# Autodesk Inventor assembly: XY Joint Left (Tulip)
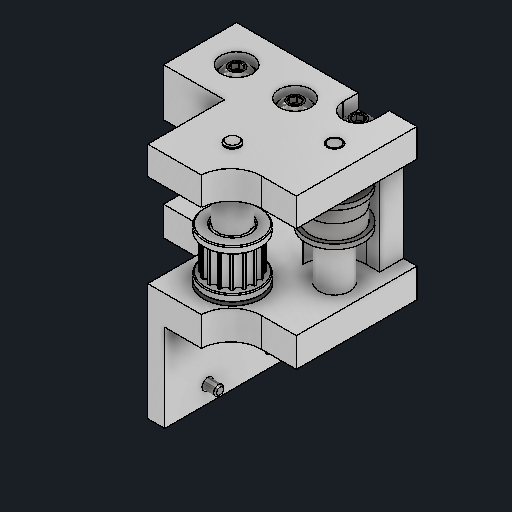
[picture p0: Inventor's stored thumbnail of the model, 512x512]
Saved by Autodesk Inventor 2026.1 (Build 301233020, 233B)
## iProperties
Created: 2025-05-24
Part Number: XY Joint Left (Tulip)
Document SubType Name: Assembly
Designer: Joshua Eah
Author: Joshua Eah
## Documents named in this file (10)
- C:\Users\JoshuaEah\Documents\GitHub\Voron-0\CAD\Tulip - Machined Parts\XY Joints\XY Joint Right\XY Joint Right (Tulip).iam
- C:\Users\JoshuaEah\Documents\GitHub\Voron-0\CAD\Tulip - Machined Parts\XY Joints\XY Joint Right\XY Joint Right Upper (Tulip).ipt
- C:\Users\JoshuaEah\Documents\GitHub\Voron-0\CAD\Tulip - Machined Parts\XY Joints\XY Joint Right\XY Joint Right Lower (Tulip).ipt
- C:\Users\JoshuaEah\Documents\GitHub\Voron-0\CAD\Master Assembly\Hardware\M3x6 BHCS.ipt
- C:\Users\JoshuaEah\Documents\GitHub\Voron-0\CAD\Master Assembly\Hardware\M3x12 BHCS.ipt
- C:\Users\JoshuaEah\Documents\GitHub\Voron-0\CAD\Master Assembly\Hardware\M2x6 FHCS.ipt
- C:\Users\JoshuaEah\Documents\GitHub\Voron-0\CAD\Tulip - Machined Parts\XY Joints\XY Joint Right\Right Idler Stack.iam
- C:\Users\JoshuaEah\Documents\GitHub\Voron-0\CAD\Tulip - Machined Parts\XY Joints\XY Joint Right\Right Pulley Stack.iam
- C:\Users\JoshuaEah\Documents\GitHub\Voron-0\CAD\Tulip - Machined Parts\XY Joints\Spacers\Joint Spacer.ipt
- C:\Users\JoshuaEah\Documents\GitHub\Voron-0\CAD\Master Assembly\Hardware\M3x25 BHCS.ipt
## Components (13 placed, 9 different names)
1. XY Joint Right Upper (Tulip):1 — Insert:1, Insert:2, Insert:9, Flush:2, Insert:11
2. XY Joint Right Lower (Tulip):1 — Insert:3, Insert:4, Insert:5, Insert:6, Insert:7, Insert:8, Flush:1, Mate:1, Mate:2, Insert:10
3. Right Idler Stack:1 [sub-assembly] — Insert:10
4. Right Pulley Stack:1 [sub-assembly] — Mate:1, Mate:2
5. M3x6 BHCS:1 — Insert:3
6. M3x12 BHCS:1 — Insert:1
7. M3x12 BHCS:2 — Insert:2
8. M3x25 BHCS:1 — Insert:11
9. M2x6 FHCS:1 — Insert:4
10. M2x6 FHCS:2 — Insert:5
11. M2x6 FHCS:3 — Insert:7
12. M2x6 FHCS:4 — Insert:6
13. Joint Spacer:1 — Insert:8, Insert:9, Flush:1, Flush:2
## Relationships (15: Insert 11, Flush 2, Mate 2)
- Insert:1: XY Joint Right Upper (Tulip):1 ↔ M3x12 BHCS:1
- Insert:2: XY Joint Right Upper (Tulip):1 ↔ M3x12 BHCS:2
- Insert:3: XY Joint Right Lower (Tulip):1 ↔ M3x6 BHCS:1
- Insert:4: XY Joint Right Lower (Tulip):1 ↔ M2x6 FHCS:1
- Insert:5: XY Joint Right Lower (Tulip):1 ↔ M2x6 FHCS:2
- Insert:6: XY Joint Right Lower (Tulip):1 ↔ M2x6 FHCS:4
- Insert:7: XY Joint Right Lower (Tulip):1 ↔ M2x6 FHCS:3
- Insert:8: XY Joint Right Lower (Tulip):1 ↔ Joint Spacer:1
- Insert:9: XY Joint Right Upper (Tulip):1 ↔ Joint Spacer:1
- Flush:1: XY Joint Right Lower (Tulip):1 ↔ Joint Spacer:1
- Flush:2: XY Joint Right Upper (Tulip):1 ↔ Joint Spacer:1
- Mate:1: XY Joint Right Lower (Tulip):1 ↔ Right Pulley Stack:1
- Mate:2: XY Joint Right Lower (Tulip):1 ↔ Right Pulley Stack:1
- Insert:10: XY Joint Right Lower (Tulip):1 ↔ Right Idler Stack:1
- Insert:11: XY Joint Right Upper (Tulip):1 ↔ M3x25 BHCS:1
